# Autodesk Inventor assembly: DC Motor Gearbox
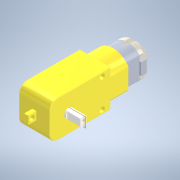
[picture p0: Inventor's stored thumbnail of the model, 180x180]
Saved by Autodesk Inventor 2020.3 (Build 243373000, 373)
## iProperties
Created: 2018-02-20
Part Number: DC Motor Gearbox
Document SubType Name: Assembly
Designer: juanp
Mass: 22.9854 g
Surface Area: 86.8564 cm^2
Volume: 22.9854 cm^3
Density: 1 g/cm^3
Sending System: SolidWorks 2018
Last Author: User
Last Saved: 2019-04-08
Author: juanp
## Documents named in this file (4)
- C:\Users\juanp\Desktop\ROBOCOL\Idea Final NAF\Motor\DC Motor Gearbox.iam
- C:\Users\juanp\Desktop\ROBOCOL\Idea Final NAF\Motor\Gearbox.ipt
- C:\Users\juanp\Desktop\ROBOCOL\Idea Final NAF\Motor\output shaft.ipt
- C:\Users\juanp\Desktop\ROBOCOL\Idea Final NAF\Motor\motor.ipt
## Components (3 placed, 3 different names)
1. Gearbox:1 — Mate:2, Angle:1, Mate:3, Flush:1, Mate:4, Angle:2
2. output shaft:1 — Flush:1, Mate:4, Angle:2
3. motor:1 — Mate:2, Angle:1, Mate:3
## Relationships (6: Mate 3, Angle 2, Flush 1)
- Mate:2: Gearbox:1 ↔ motor:1
- Angle:1 (0 deg): Gearbox:1 ↔ motor:1
- Mate:3: Gearbox:1 ↔ motor:1
- Flush:1 (-9 mm): Gearbox:1 ↔ output shaft:1
- Mate:4: Gearbox:1 ↔ output shaft:1
- Angle:2 (0 deg): Gearbox:1 ↔ output shaft:1
